# Autodesk Inventor assembly: Сборка
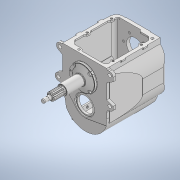
[picture p0: Inventor's stored thumbnail of the model, 180x180]
Saved by Autodesk Inventor 2021 (Build 250183000, 183)
## iProperties
Created: 2021-04-26
Part Number: Сборка
Document SubType Name: Assembly
Designer: Данил
Author: Данил
## Documents named in this file (9)
- C:\Users\Данил\Desktop\Коробка передач\Детали\Сборка.iam
- C:\Users\Данил\Desktop\Коробка передач\Детали\66-67. Картер коробки передач.ipt
- C:\Users\Данил\Desktop\Коробка передач\Детали\74. Вал первичный в сборе.iam
- C:\Users\Данил\Desktop\Коробка передач\Детали\Подшипник 180209 ГОСТ 8882-75.ipt
- C:\Users\Данил\Desktop\Коробка передач\Детали\65. Кольцо упорное подшипника.ipt
- C:\Users\Данил\Desktop\Коробка передач\Детали\76. Гайка первичного вала.ipt
- C:\Users\Данил\Desktop\Коробка передач\Детали\75. Прокладка крышки.ipt
- C:\Users\Данил\Desktop\Коробка передач\Детали\73. Крышка подшипника.ipt
- C:\Users\Данил\Desktop\Коробка передач\Детали\34. Скоба оттяжной пружины муфты.ipt
## Components (8 placed, 8 different names)
1. 66-67. Картер коробки передач:1 — Совмещение:5, Совмещение:8, Совмещение:9, Совмещение:10, Совмещение:11, Совмещение:14, Совмещение:15
2. 74. Вал первичный в сборе:1 [sub-assembly] — Совмещение:1, Совмещение:2, Совмещение:5, Совмещение:6, Совмещение:13
3. Подшипник 180000 ГОСТ 8882-75 180209:1 — Совмещение:1, Совмещение:2, Совмещение:3, Совмещение:4, Совмещение:7
4. 65. Кольцо упорное подшипника:1 — Совмещение:3, Совмещение:4, Совмещение:12
5. 76. Гайка первичного вала:1 — Совмещение:6, Совмещение:7
6. 75. Прокладка крышки:1 — Совмещение:8, Совмещение:9, Совмещение:10, Совмещение:11, Совмещение:12, Совмещение:16
7. 73. Крышка подшипника:1 — Совмещение:13, Совмещение:14, Совмещение:15, Совмещение:16, Совмещение:17, Угол:1, Совмещение:18
8. 34. Скоба оттяжной пружины муфты:1 — Совмещение:17, Угол:1, Совмещение:18
## Relationships (19: Mate 18, Angle 1)
- Совмещение:1 [Mate]: 74. Вал первичный в сборе:1 ↔ Подшипник 180000 ГОСТ 8882-75 180209:1
- Совмещение:2 [Mate]: 74. Вал первичный в сборе:1 ↔ Подшипник 180000 ГОСТ 8882-75 180209:1
- Совмещение:3 [Mate]: Подшипник 180000 ГОСТ 8882-75 180209:1 ↔ 65. Кольцо упорное подшипника:1
- Совмещение:4 [Mate]: Подшипник 180000 ГОСТ 8882-75 180209:1 ↔ 65. Кольцо упорное подшипника:1
- Совмещение:5 [Mate]: 66-67. Картер коробки передач:1 ↔ 74. Вал первичный в сборе:1
- Совмещение:6 [Mate]: 74. Вал первичный в сборе:1 ↔ 76. Гайка первичного вала:1
- Совмещение:7 [Mate]: Подшипник 180000 ГОСТ 8882-75 180209:1 ↔ 76. Гайка первичного вала:1
- Совмещение:8 [Mate]: 66-67. Картер коробки передач:1 ↔ 75. Прокладка крышки:1
- Совмещение:9 [Mate]: 66-67. Картер коробки передач:1 ↔ 75. Прокладка крышки:1
- Совмещение:10 [Mate]: 66-67. Картер коробки передач:1 ↔ 75. Прокладка крышки:1
- Совмещение:11 [Mate]: 66-67. Картер коробки передач:1 ↔ 75. Прокладка крышки:1
- Совмещение:12 [Mate]: 65. Кольцо упорное подшипника:1 ↔ 75. Прокладка крышки:1
- Совмещение:13 [Mate]: 74. Вал первичный в сборе:1 ↔ 73. Крышка подшипника:1
- Совмещение:14 [Mate]: 66-67. Картер коробки передач:1 ↔ 73. Крышка подшипника:1
- Совмещение:15 [Mate]: 66-67. Картер коробки передач:1 ↔ 73. Крышка подшипника:1
- Совмещение:16 [Mate]: 75. Прокладка крышки:1 ↔ 73. Крышка подшипника:1
- Совмещение:17 [Mate]: 73. Крышка подшипника:1 ↔ 34. Скоба оттяжной пружины муфты:1
- Угол:1 [Angle] (0 deg): 73. Крышка подшипника:1 ↔ 34. Скоба оттяжной пружины муфты:1
- Совмещение:18 [Mate]: 73. Крышка подшипника:1 ↔ 34. Скоба оттяжной пружины муфты:1
